# Autodesk Inventor assembly: RightCover
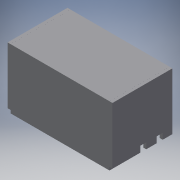
[picture p0: Inventor's stored thumbnail of the model, 180x180]
Saved by Autodesk Inventor 2016 (Build 200138000, 138)
## iProperties
Created: 2016-05-30
Part Number: RightCover
Document SubType Name: Assembly
Designer: cutrones
Author: cutrones
## Documents named in this file (5)
- U:\MotorCovers\RightCover\RightCover.iam
- U:\MotorCovers\RightCover\OutsideRWall.ipt
- U:\MotorCovers\RightCover\TopRWall.ipt
- U:\MotorCovers\RightCover\InsideRWall.ipt
- U:\MotorCovers\RightCover\SideRWall.ipt
## Components (5 placed, 4 different names)
1. OutsideRWall:1 — Flush:1, Flush:2, Flush:3, Flush:4, Flush:5, Mate:1, Flush:9
2. TopRWall:1 — Flush:4, Flush:5, Mate:1, Flush:6, Flush:7, Mate:2, Mate:3, Flush:8, Flush:10
3. InsideRWall:1 — Flush:6, Flush:7, Mate:2, Mate:4, Flush:11
4. SideRWall:1 — Mate:4, Flush:10, Flush:11
5. SideRWall:2 — Mate:3, Flush:8, Flush:9
## Relationships (15: Flush 11, Mate 4)
- Flush:1: OutsideRWall:1
- Flush:2: OutsideRWall:1
- Flush:3: OutsideRWall:1
- Flush:4: OutsideRWall:1 ↔ TopRWall:1
- Flush:5: OutsideRWall:1 ↔ TopRWall:1
- Mate:1: OutsideRWall:1 ↔ TopRWall:1
- Flush:6: TopRWall:1 ↔ InsideRWall:1
- Flush:7: TopRWall:1 ↔ InsideRWall:1
- Mate:2: TopRWall:1 ↔ InsideRWall:1
- Mate:3: TopRWall:1 ↔ SideRWall:2
- Flush:8: TopRWall:1 ↔ SideRWall:2
- Flush:9: OutsideRWall:1 ↔ SideRWall:2
- Mate:4: InsideRWall:1 ↔ SideRWall:1
- Flush:10: TopRWall:1 ↔ SideRWall:1
- Flush:11: InsideRWall:1 ↔ SideRWall:1
